# Autodesk Inventor assembly: auth panel assembly
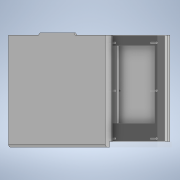
[picture p0: Inventor's stored thumbnail of the model, 180x180]
Saved by Autodesk Inventor 2022 (Build 260153000, 153)
## iProperties
Created: 2022-06-08
Part Number: auth panel assembly
Document SubType Name: Assembly
Designer: alecw
Author: alecw
## Documents named in this file (10)
- W:\My Drive\Coding and Projects\smart home\smart-deadbolt\3D Modelling\auth panel assembly.iam
- W:\My Drive\Coding and Projects\smart home\smart-deadbolt\3D Modelling\auth panel face plate seal.ipt
- W:\My Drive\Coding and Projects\smart home\smart-deadbolt\3D Modelling\auth panel cover.ipt
- W:\My Drive\Coding and Projects\smart home\smart-deadbolt\3D Modelling\auth panel face plate.ipt
- W:\My Drive\Coding and Projects\smart home\smart-deadbolt\3D Modelling\keypad and cover.iam
- W:\My Drive\Coding and Projects\smart home\smart-deadbolt\3D Modelling\fingerprint sensor.ipt
- W:\My Drive\Coding and Projects\smart home\smart-deadbolt\3D Modelling\1x3 button assembly.iam
- W:\My Drive\Coding and Projects\smart home\smart-deadbolt\3D Modelling\authentication panel.ipt
- W:\My Drive\Coding and Projects\smart home\smart-deadbolt\3D Modelling\fingerprint sensor seal.ipt
- W:\My Drive\Coding and Projects\smart home\smart-deadbolt\3D Modelling\rfid cover.ipt
## Components (9 placed, 9 different names)
1. auth panel face plate seal:1 — Mate:1, Flush:1, Flush:2, Mate:2, Mate:14
2. auth panel cover:1 — Flush:5, Cylindrical:1
3. auth panel face plate:1 — Mate:2, Flush:3, Flush:4, Mate:3, Mate:6, Mate:7, Flush:6
4. keypad and cover:1 [sub-assembly] — Mate:6, Mate:7, Mate:13
5. authentication panel:1 — Mate:1, Flush:1, Flush:2, Flush:3, Flush:4, Flush:5, Mate:4, Mate:5, Mate:10, Mate:11, Mate:12, Mate:13, Flush:7, Flush:8, Mate:15, Mate:16, Mate:17, Cylindrical:1
6. fingerprint sensor:1 — Flush:6, Mate:12
7. 1x3 button assembly:1 [sub-assembly] — Mate:3, Mate:4, Mate:5
8. fingerprint sensor seal:1 — Mate:10, Mate:11
9. rfid cover:1 — Flush:7, Flush:8, Mate:14
## Relationships (24: Mate 15, Flush 8, CylindricalJoint 1)
- Mate:1: auth panel face plate seal:1 ↔ authentication panel:1
- Flush:1: auth panel face plate seal:1 ↔ authentication panel:1
- Flush:2: auth panel face plate seal:1 ↔ authentication panel:1
- Mate:2: auth panel face plate seal:1 ↔ auth panel face plate:1
- Flush:3: auth panel face plate:1 ↔ authentication panel:1
- Flush:4: auth panel face plate:1 ↔ authentication panel:1
- Flush:5: auth panel cover:1 ↔ authentication panel:1
- Mate:3: auth panel face plate:1 ↔ 1x3 button assembly:1
- Mate:4 (0.25 mm): authentication panel:1 ↔ 1x3 button assembly:1
- Mate:5 (0.25 mm): authentication panel:1 ↔ 1x3 button assembly:1
- Mate:6: auth panel face plate:1 ↔ keypad and cover:1
- Mate:7: auth panel face plate:1 ↔ keypad and cover:1
- Flush:6: auth panel face plate:1 ↔ fingerprint sensor:1
- Mate:10: authentication panel:1 ↔ fingerprint sensor seal:1
- Mate:11: authentication panel:1 ↔ fingerprint sensor seal:1
- Mate:12: authentication panel:1 ↔ fingerprint sensor:1
- Mate:13: keypad and cover:1 ↔ authentication panel:1
- Flush:7: authentication panel:1 ↔ rfid cover:1
- Flush:8: authentication panel:1 ↔ rfid cover:1
- Mate:14: auth panel face plate seal:1 ↔ rfid cover:1
- Mate:15: authentication panel:1
- Mate:16: authentication panel:1
- Mate:17: authentication panel:1
- Cylindrical:1: auth panel cover:1 ↔ authentication panel:1
